# Autodesk Inventor assembly: single-elemnt -assembly
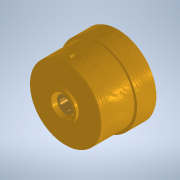
[picture p0: Inventor's stored thumbnail of the model, 180x180]
Saved by Autodesk Inventor 2022 (Build 260153000, 153)
## iProperties
Created: 2021-08-02
Part Number: single-elemnt -assembly
Document SubType Name: Assembly
Designer: user
Author: user
## Documents named in this file (4)
- C:\Users\user\Documents\School work\Fourth Year\Manufacturing Technology I\Coaxial-swirl-injector\single-elemnt -assembly.iam
- C:\Users\user\Documents\School work\Fourth Year\Manufacturing Technology I\Coaxial-swirl-injector\base_single.ipt
- C:\Users\user\Documents\School work\Fourth Year\Manufacturing Technology I\Coaxial-swirl-injector\injector assembly.iam
- C:\Users\user\Documents\School work\Fourth Year\Manufacturing Technology I\Coaxial-swirl-injector\separator_single.ipt
## Components (3 placed, 3 different names)
1. base_single:1 — Mate:1, Mate:2, Mate:3, Mate:4, Mate:5, Mate:6, Mate:7
2. injector assembly:1 [sub-assembly] — Mate:1, Mate:2, Mate:3, Mate:4, Mate:5
3. separator_single:1 — Mate:6, Mate:7
## Relationships (7: Mate 7)
- Mate:1: base_single:1 ↔ injector assembly:1
- Mate:2: base_single:1 ↔ injector assembly:1
- Mate:3: base_single:1 ↔ injector assembly:1
- Mate:4: base_single:1 ↔ injector assembly:1
- Mate:5: base_single:1 ↔ injector assembly:1
- Mate:6: base_single:1 ↔ separator_single:1
- Mate:7: base_single:1 ↔ separator_single:1
